# Autodesk Inventor assembly: Assembly_revised
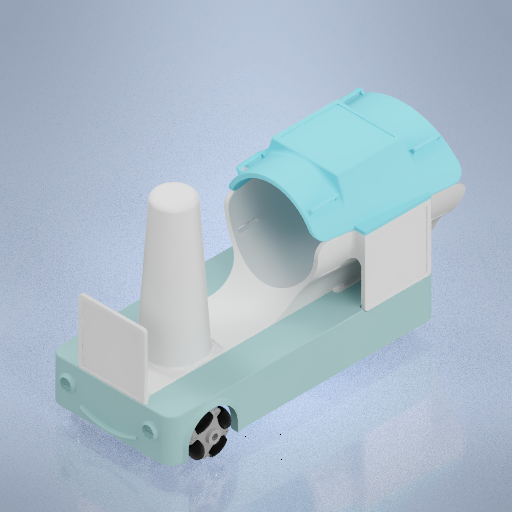
[picture p0: Inventor's stored thumbnail of the model, 512x512]
Saved by Autodesk Inventor 2025 (Build 290162000, 162)
## iProperties
Created: 2024-06-29
Part Number: Assembly_revised
Document SubType Name: Assembly
Designer: Pintu
Author: Pintu
## Documents named in this file (6)
- D:\CMC\my_inventor\ArmBo_v2\wearable\Assembly_revised.iam
- D:\CMC\my_inventor\ArmBo_v2\wearable\chasis.ipt
- D:\CMC\my_inventor\ArmBo_v2\wearable\wearable.ipt
- D:\CMC\my_inventor\ArmBo_v2\wearable\aruco_top_marker.ipt
- D:\CMC\my_inventor\ArmBo_v2\wheels\omniwheel_38mm\omniwheel_38mm\wheel_38mm_assembly.iam
- D:\CMC\my_inventor\ArmBo_v2\wheels\omniwheel_38mm\omniwheel_38mm\wheel_holder_2.ipt
## Components (9 placed, 5 different names)
1. chasis:1 — Flush:1, Flush:2, Flush:3, Mate:4, Mate:5, Mate:6, Mate:8, Mate:9, Mate:10, Mate:13, Mate:14, Mate:15
2. wearable:1 — Mate:1, Mate:2, Mate:3, Flush:1, Flush:2, Flush:3
3. aruco_top_marker:1 — Mate:1, Mate:2, Mate:3
4. wheel_38mm_assembly:1 [sub-assembly] — Mate:16, Mate:17
5. wheel_38mm_assembly:2 [sub-assembly] — Mate:11, Mate:12
6. wheel_38mm_assembly:3 [sub-assembly] — Mate:7, Mate:18
7. wheel_holder_2:1 — Mate:4, Mate:5, Mate:6, Mate:7, Mate:18
8. wheel_holder_2:2 — Mate:13, Mate:14, Mate:15, Mate:16, Mate:17
9. wheel_holder_2:3 — Mate:8, Mate:9, Mate:10, Mate:11, Mate:12
## Relationships (21: Mate 18, Flush 3)
- Mate:1 (0.5 mm): wearable:1 ↔ aruco_top_marker:1
- Mate:2 (0.5 mm): wearable:1 ↔ aruco_top_marker:1
- Mate:3: wearable:1 ↔ aruco_top_marker:1
- Flush:1: chasis:1 ↔ wearable:1
- Flush:2 (1 mm): chasis:1 ↔ wearable:1
- Flush:3 (121 mm): chasis:1 ↔ wearable:1
- Mate:4: chasis:1 ↔ wheel_holder_2:1
- Mate:5: chasis:1 ↔ wheel_holder_2:1
- Mate:6: chasis:1 ↔ wheel_holder_2:1
- Mate:7: wheel_38mm_assembly:3 ↔ wheel_holder_2:1
- Mate:8: chasis:1 ↔ wheel_holder_2:3
- Mate:9: chasis:1 ↔ wheel_holder_2:3
- Mate:10: chasis:1 ↔ wheel_holder_2:3
- Mate:11: wheel_38mm_assembly:2 ↔ wheel_holder_2:3
- Mate:12: wheel_38mm_assembly:2 ↔ wheel_holder_2:3
- Mate:13: chasis:1 ↔ wheel_holder_2:2
- Mate:14: chasis:1 ↔ wheel_holder_2:2
- Mate:15: chasis:1 ↔ wheel_holder_2:2
- Mate:16: wheel_38mm_assembly:1 ↔ wheel_holder_2:2
- Mate:17: wheel_38mm_assembly:1 ↔ wheel_holder_2:2
- Mate:18: wheel_38mm_assembly:3 ↔ wheel_holder_2:1
